# Autodesk Inventor assembly: Lead_Screw_Assy
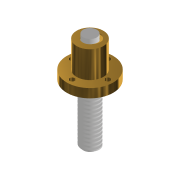
[picture p0: Inventor's stored thumbnail of the model, 180x180]
Saved by Autodesk Inventor 2020 (Build 240168000, 168)
## iProperties
Created: 2023-03-22
Part Number: Lead_Screw_Assy
Document SubType Name: Assembly
Designer: ADMIN
Author: ADMIN
## Documents named in this file (3)
- D:\My_Thoughts\Rough\Lead_Screw_Assy.iam
- D:\My_Thoughts\Rough\LeadScrew.ipt
- D:\My_Thoughts\Rough\TR-20x4 nut.ipt
## Components (2 placed, 2 different names)
1. LeadScrew:1 — Mate:1, Tangent:1
2. TR-20x4 nut:1 — Mate:1, Tangent:1
## Relationships (2: Mate 1, Tangent 1)
- Mate:1: LeadScrew:1 ↔ TR-20x4 nut:1
- Tangent:1: LeadScrew:1 ↔ TR-20x4 nut:1
